# Autodesk Inventor assembly: RS-775GM_004GH
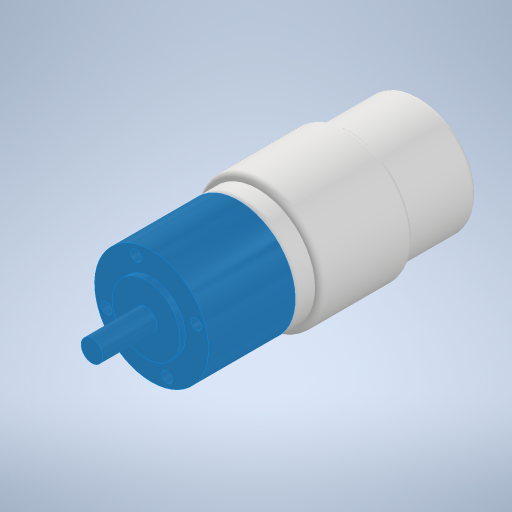
[picture p0: Inventor's stored thumbnail of the model, 512x512]
Saved by Autodesk Inventor 2024.1 (Build 281209000, 209)
## iProperties
Created: 2022-11-14
Part Number: RS-775GM_004GH
Document SubType Name: Assembly
Designer: blueh
Author: blueh
## Documents named in this file (3)
- C:\Users\haruy\OneDrive - Kyushu University\cad\000_parts\モーター\RS-775GM_004GH.iam
- C:\Users\haruy\OneDrive - Kyushu University\cad\000_parts\モーター\RS-775GM.ipt
- C:\Users\haruy\OneDrive - Kyushu University\cad\000_parts\モーター\RS-775GM_004GH_sn.ipt
## Components (2 placed, 2 different names)
1. RS-775GM:1
2. RS-775GM_004GH_sn:1
## Relationships (1: Insert 1)
- [Insert]: RS-775GM:1 ↔ RS-775GM_004GH_sn:1
